# Autodesk Inventor assembly: wheel_pair
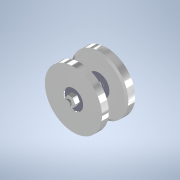
[picture p0: Inventor's stored thumbnail of the model, 180x180]
Saved by Autodesk Inventor 2020.3 (Build 243373000, 373)
## iProperties
Created: 2021-03-25
Part Number: wheel_pair
Document SubType Name: Assembly
Designer: patry
Mass: 73.5609 g
Surface Area: 155.822 cm^2
Volume: 27.2448 cm^3
Density: 2.7 g/cm^3
Author: patry
## Documents named in this file (5)
- C:\Users\patry\Desktop\Semestr 7\Inzynierka\Projekt inventor\Ariadna_inzynierka\Workspaces\Obszar roboczy\Obszar roboczy\Naped\Kola\wheel_pair.iam
- C:\Users\patry\Desktop\Semestr 7\Inzynierka\Projekt inventor\Ariadna_inzynierka\Workspaces\Obszar roboczy\Obszar roboczy\Naped\Kola\single_wheel.iam
- C:\Users\patry\Desktop\Semestr 7\Inzynierka\Projekt inventor\Ariadna_inzynierka\Workspaces\Obszar roboczy\Obszar roboczy\Naped\Sruby\M5_nut_5mm.ipt
- C:\Users\patry\Desktop\Semestr 7\Inzynierka\Projekt inventor\Ariadna_inzynierka\Workspaces\Obszar roboczy\Obszar roboczy\Naped\Sruby\M5_40_shaft.ipt
- M5_shaft.ipt
## Components (7 placed, 3 different names)
1. single_wheel:1 [sub-assembly] — Zestawiające:1, Zestawiające:2, Zestawiające:6, Mate:11, Zestawiające:15
2. single_wheel:2 [sub-assembly] — Zestawiające:1, Zestawiające:2, Zestawiające:9, Zestawiające:12, Równoległe:1, Zestawiające:17
3. M5_nut_5mm:1 — Zestawiające:6, Zestawiające:15
4. M5_nut_5mm:3 — Zestawiające:9, Zestawiające:13
5. M5_nut_5mm:4 — Mate:11, Zestawiające:14
6. M5_shaft:1 — Zestawiające:12, Zestawiające:13, Zestawiające:14, Równoległe:1, Zestawiające:16
7. M5_nut_5mm:5 — Zestawiające:16, Zestawiające:17
## Relationships (12: Mate 11, Flush 1)
- Zestawiające:1 [Mate] (15 mm): single_wheel:1 ↔ single_wheel:2
- Zestawiające:2 [Mate]: single_wheel:1 ↔ single_wheel:2
- Zestawiające:6 [Mate]: single_wheel:1 ↔ M5_nut_5mm:1
- Zestawiające:9 [Mate]: single_wheel:2 ↔ M5_nut_5mm:3
- Mate:11: single_wheel:1 ↔ M5_nut_5mm:4
- Zestawiające:12 [Mate]: single_wheel:2 ↔ M5_shaft:1
- Zestawiające:13 [Mate]: M5_nut_5mm:3 ↔ M5_shaft:1
- Zestawiające:14 [Mate]: M5_nut_5mm:4 ↔ M5_shaft:1
- Zestawiające:15 [Mate]: single_wheel:1 ↔ M5_nut_5mm:1
- Równoległe:1 [Flush] (5.5 mm): single_wheel:2 ↔ M5_shaft:1
- Zestawiające:16 [Mate]: M5_shaft:1 ↔ M5_nut_5mm:5
- Zestawiające:17 [Mate]: single_wheel:2 ↔ M5_nut_5mm:5
